# Autodesk Inventor assembly: Chassis
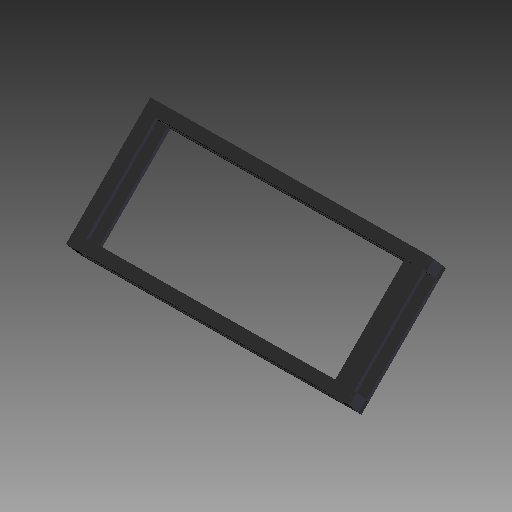
[picture p0: Inventor's stored thumbnail of the model, 512x512]
Saved by Autodesk Inventor 2017 SP1 (Build 210196100, 196)
## iProperties
Created: 2017-08-21
Part Number: Chassis
Document SubType Name: Assembly
Designer: Zach
Author: Zach
## Documents named in this file (5)
- C:\Users\Zach\Documents\GitHub\tr1\src\Body\Chest Assembly\Chassis\Chassis.iam
- C:\Users\Zach\Documents\GitHub\tr1\src\Body\Chest Assembly\Chassis\C008.ipt
- C:\Users\Zach\Documents\GitHub\tr1\src\Body\Chest Assembly\Chassis\C010.ipt
- C:\Users\Zach\Documents\GitHub\tr1\src\Body\Chest Assembly\Chassis\C011.ipt
- C:\Users\Zach\Documents\GitHub\tr1\src\Body\Chest Assembly\Chassis\C014.ipt
## Components (13 placed, 4 different names)
1. C008:1 — Mate:1, Flush:1, Flush:2, Flush:4, Mate:2, Mate:13
2. C010:1 — Mate:1, Flush:1, Flush:2, Flush:3, Flush:9, Flush:10, Flush:11, Mate:6
3. C011:1 — Flush:3, Flush:4, Mate:2, Flush:5, Flush:6, Mate:3, Flush:7
4. C014:1 — Mate:19, Flush:20, Mate:20
5. C008:2 — Flush:5, Flush:6, Mate:3, Flush:8, Mate:4
6. C010:2 — Flush:7, Flush:8, Mate:4, Mate:5, Flush:13
7. C011:2 — Flush:9, Mate:5, Flush:12, Flush:14, Mate:7
8. C008:3 — Flush:13, Flush:14, Mate:7, Mate:19
9. C008:4 — Flush:10, Flush:11, Mate:6, Flush:12, Flush:18, Flush:19
10. C010:3 — Mate:9, Mate:11, Flush:18, Mate:13
11. C011:3 — Mate:11, Mate:12
12. C010:4 — Mate:10, Mate:12
13. C011:4 — Mate:9, Mate:10, Flush:19, Flush:20, Mate:20
## Relationships (35: Flush 20, Mate 15)
- Mate:1: C008:1 ↔ C010:1
- Flush:1: C008:1 ↔ C010:1
- Flush:2: C008:1 ↔ C010:1
- Flush:3: C010:1 ↔ C011:1
- Flush:4: C008:1 ↔ C011:1
- Mate:2: C008:1 ↔ C011:1
- Flush:5: C011:1 ↔ C008:2
- Flush:6: C011:1 ↔ C008:2
- Mate:3: C011:1 ↔ C008:2
- Flush:7: C011:1 ↔ C010:2
- Flush:8: C008:2 ↔ C010:2
- Mate:4: C008:2 ↔ C010:2
- Flush:9: C010:1 ↔ C011:2
- Mate:5: C010:2 ↔ C011:2
- Flush:10: C010:1 ↔ C008:4
- Flush:11: C010:1 ↔ C008:4
- Mate:6: C010:1 ↔ C008:4
- Flush:12: C011:2 ↔ C008:4
- Flush:13: C010:2 ↔ C008:3
- Flush:14: C011:2 ↔ C008:3
- Mate:7: C011:2 ↔ C008:3
- [Flush]: C010:3 ↔ C011:3
- [Flush]: C011:3 ↔ C010:4
- [Flush]: C010:3 ↔ C011:4
- [Mate]: C010:4 ↔ C011:4
- Mate:9: C010:3 ↔ C011:4
- Mate:10: C010:4 ↔ C011:4
- Mate:11: C010:3 ↔ C011:3
- Mate:12: C011:3 ↔ C010:4
- Flush:18: C008:4 ↔ C010:3
- Flush:19: C008:4 ↔ C011:4
- Mate:13: C008:1 ↔ C010:3
- Mate:19 (28 mm): C014:1 ↔ C008:3
- Flush:20: C014:1 ↔ C011:4
- Mate:20: C014:1 ↔ C011:4
## Named parameters: d22_d3 = 0 mm, d23_d9 = 0 mm, d24_d12 = 0 mm, d25_d14 = 0 mm
